# Autodesk Inventor assembly: Assembly1
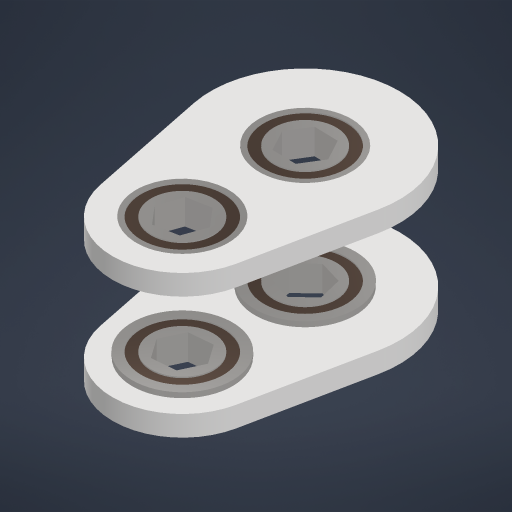
[picture p0: Inventor's stored thumbnail of the model, 512x512]
Saved by Autodesk Inventor 2024.4 (Build 284460000, 460)
## iProperties
Created: 2026-06-11
Part Number: Assembly1
Document SubType Name: Assembly
Designer: hs4ho
Author: hs4ho
## Documents named in this file (3)
- C:\Users\hs4ho\OneDrive\Documents\GitHub\2026-2027-DesignTraining\DeanS\Assembly1.iam
- C:\Users\hs4ho\OneDrive\Documents\GitHub\2026-2027-DesignTraining\DeanS\DTraining2_001_E1Base.ipt
- C:\Users\hs4ho\OneDrive\Documents\GitHub\2026-2027-DesignTraining\COTS Library\Motion\Bearings\COTS_WCP-0783_1.125ODHexBearing.ipt
## Components (6 placed, 2 different names)
1. DTraining2_001_E1Base:1 — Mate:1, Mate:2, Mate:3, Mate:4, Mate:5, Mate:6
2. DTraining2_001_E1Base:2 — Mate:1, Mate:2, Mate:7, Mate:8, Mate:9, Mate:10
3. COTS_WCP-0783_1.125ODHexBearing:1 — Mate:3, Mate:4
4. COTS_WCP-0783_1.125ODHexBearing:2 — Mate:5, Mate:6
5. COTS_WCP-0783_1.125ODHexBearing:3 — Mate:7, Mate:8
6. COTS_WCP-0783_1.125ODHexBearing:4 — Mate:9, Mate:10
## Relationships (10: Mate 10)
- Mate:1: DTraining2_001_E1Base:1 ↔ DTraining2_001_E1Base:2
- Mate:2: DTraining2_001_E1Base:1 ↔ DTraining2_001_E1Base:2
- Mate:3: DTraining2_001_E1Base:1 ↔ COTS_WCP-0783_1.125ODHexBearing:1
- Mate:4: DTraining2_001_E1Base:1 ↔ COTS_WCP-0783_1.125ODHexBearing:1
- Mate:5: DTraining2_001_E1Base:1 ↔ COTS_WCP-0783_1.125ODHexBearing:2
- Mate:6: DTraining2_001_E1Base:1 ↔ COTS_WCP-0783_1.125ODHexBearing:2
- Mate:7: DTraining2_001_E1Base:2 ↔ COTS_WCP-0783_1.125ODHexBearing:3
- Mate:8: DTraining2_001_E1Base:2 ↔ COTS_WCP-0783_1.125ODHexBearing:3
- Mate:9: DTraining2_001_E1Base:2 ↔ COTS_WCP-0783_1.125ODHexBearing:4
- Mate:10: DTraining2_001_E1Base:2 ↔ COTS_WCP-0783_1.125ODHexBearing:4
